# Autodesk Inventor assembly: FullCanAssembly
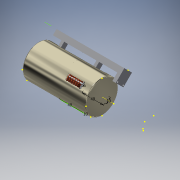
[picture p0: Inventor's stored thumbnail of the model, 180x180]
Saved by Autodesk Inventor 2017.3 (Build 213256000, 256)
## iProperties
Created: 2018-05-23
Part Number: FullCanAssembly
Document SubType Name: Assembly
Designer: Mac
Author: Mac
## Documents named in this file (18)
- C:\Users\Mac\Desktop\UNR Coltrims\eGun Final Design\FullCanAssembly.iam
- C:\Users\Mac\Desktop\UNR Coltrims\eGun Final Design\Ceramic Support.ipt
- C:\Users\Mac\Desktop\UNR Coltrims\eGun Final Design\InnerSleeveBack.ipt
- C:\Users\Mac\Desktop\UNR Coltrims\eGun Final Design\InnerSleeveFront.ipt
- C:\Users\Mac\Desktop\UNR Coltrims\eGun Final Design\13mm Ceramic Spacer.ipt
- C:\Users\Mac\Desktop\UNR Coltrims\eGun Final Design\Pulser Plate.ipt
- C:\Users\Mac\Desktop\UNR Coltrims\eGun Final Design\19mm Ceramic Spacer.ipt
- C:\Users\Mac\Desktop\UNR Coltrims\eGun Final Design\1mm Electrode.ipt
- C:\Users\Mac\Desktop\UNR Coltrims\eGun Final Design\20mm Ceramic Spacer.ipt
- C:\Users\Mac\Desktop\UNR Coltrims\eGun Final Design\3mm Ceramic Spacer.ipt
- C:\Users\Mac\Desktop\UNR Coltrims\eGun Final Design\uMetal Can.ipt
- C:\Users\Mac\Desktop\UNR Coltrims\eGun Final Design\uMetal Can Backside.ipt
- C:\Users\Mac\Desktop\UNR Coltrims\eGun Final Design\4.5mm Ceramic Spacer.ipt
- C:\Users\Mac\Desktop\UNR Coltrims\eGun Final Design\Cathode\Cathode Assembly.iam
- C:\Users\Mac\Desktop\UNR Coltrims\eGun Final Design\Sleeve Endcap.ipt
- C:\Users\Mac\Desktop\UNR Coltrims\eGun Final Design\body rod.ipt
- C:\Users\Mac\Desktop\UNR Coltrims\eGun Final Design\L bracket.ipt
- C:\Users\Mac\Desktop\UNR Coltrims\eGun Final Design\holder square.ipt
## Components (77 placed, 17 different names)
1. Ceramic Support:1 — Mate:1, Mate:2, Mate:3, Mate:4, Mate:5, Mate:6, Mate:7, Mate:8, Mate:9, Mate:16, Mate:17, Mate:19, Mate:20, Mate:22, Mate:23, Mate:24, Mate:25, Mate:26, Mate:27, Mate:34, Mate:35, Mate:37, Mate:38, Mate:39, Mate:40, Mate:41, Mate:42, Mate:49, Mate:50, Mate:52, Mate:53, Mate:54, Mate:55, Mate:56, Mate:57, Mate:64, Mate:65, Mate:67, Mate:68, Mate:69, Mate:70, Mate:71, Mate:72, Mate:79, Mate:80, Mate:82, Mate:83, Mate:84, Mate:85, Mate:86, Mate:87, Mate:94, Mate:95, Mate:97, Mate:98, Mate:99, Mate:100, Mate:101, Mate:102, Mate:109, Mate:110, Mate:112, Mate:113, Mate:114, Mate:115, Mate:116, Mate:117, Mate:124, Mate:125, Mate:127, Mate:128, Mate:129, Mate:130, Mate:131, Mate:132, Mate:139, Mate:140, Mate:142, Mate:143, Mate:144
2. InnerSleeveBack:1 — Mate:145, Mate:146, Mate:147
3. InnerSleeveFront:1 — Mate:1, Mate:2, Mate:3, Mate:10, Mate:11, Mate:12, Mate:13, Mate:14, Mate:15, Mate:148, Mate:149, Mate:150, Mate:151, Flush:1, Flush:2, Flush:3, Flush:4, Mate:152, Mate:153, Mate:161
4. 13mm Ceramic Spacer:1 — Mate:4, Mate:14
5. 13mm Ceramic Spacer:2 — Mate:5, Mate:10
6. 13mm Ceramic Spacer:3 — Mate:6, Mate:11, Mate:18
7. 13mm Ceramic Spacer:4 — Mate:7, Mate:12
8. 13mm Ceramic Spacer:5 — Mate:8, Mate:13
9. 13mm Ceramic Spacer:6 — Mate:9, Mate:15, Mate:21
10. Pulser Plate:1 — Mate:16, Mate:17, Mate:18, Mate:31, Mate:32, Mate:33
11. Pulser Plate:2 — Mate:19, Mate:20, Mate:21, Mate:28, Mate:29, Mate:30
12. 19mm Ceramic Spacer:1 — Mate:22, Mate:29
13. 19mm Ceramic Spacer:2 — Mate:23, Mate:28
14. 19mm Ceramic Spacer:3 — Mate:24, Mate:33, Mate:36
15. 19mm Ceramic Spacer:4 — Mate:25, Mate:32
16. 19mm Ceramic Spacer:5 — Mate:26, Mate:31
17. 19mm Ceramic Spacer:6 — Mate:27, Mate:30
18. 1mm Electrode:1 — Mate:64, Mate:65, Mate:66, Mate:73, Mate:74, Mate:75, Mate:76, Mate:77, Mate:78
19. 1mm Electrode:2 — Mate:34, Mate:35, Mate:36, Mate:43, Mate:44, Mate:45, Mate:46, Mate:47, Mate:48
20. 1mm Electrode:3 — Mate:79, Mate:80, Mate:81, Mate:88, Mate:89, Mate:90, Mate:91, Mate:92, Mate:93
21. 1mm Electrode:4 — Mate:49, Mate:50, Mate:51, Mate:58, Mate:59, Mate:60, Mate:61, Mate:62, Mate:63
22. 1mm Electrode:5 — Mate:109, Mate:110, Mate:111, Mate:118, Mate:119, Mate:120, Mate:121, Mate:122, Mate:123
23. 1mm Electrode:6 — Mate:94, Mate:95, Mate:96, Mate:103, Mate:104, Mate:105, Mate:106, Mate:107, Mate:108
24. 20mm Ceramic Spacer:1 — Mate:42, Mate:48
25. 20mm Ceramic Spacer:2 — Mate:41, Mate:47
26. 20mm Ceramic Spacer:3 — Mate:40, Mate:46
27. 20mm Ceramic Spacer:4 — Mate:39, Mate:45
28. 20mm Ceramic Spacer:5 — Mate:38, Mate:44
29. 20mm Ceramic Spacer:6 — Mate:37, Mate:43, Mate:51
30. 3mm Ceramic Spacer:1 — Mate:52, Mate:61
31. 3mm Ceramic Spacer:2 — Mate:53, Mate:62
32. 3mm Ceramic Spacer:3 — Mate:54, Mate:63
33. 3mm Ceramic Spacer:4 — Mate:55, Mate:58
34. 3mm Ceramic Spacer:5 — Mate:56, Mate:59
35. 3mm Ceramic Spacer:6 — Mate:57, Mate:60, Mate:66
36. 3mm Ceramic Spacer:7 — Mate:87, Mate:91
37. 3mm Ceramic Spacer:8 — Mate:86, Mate:90
38. 3mm Ceramic Spacer:9 — Mate:85, Mate:89
39. 3mm Ceramic Spacer:10 — Mate:84, Mate:88
40. 3mm Ceramic Spacer:11 — Mate:83, Mate:93
41. 3mm Ceramic Spacer:12 — Mate:82, Mate:92, Mate:96
42. 3mm Ceramic Spacer:13 — Mate:102, Mate:107
43. 3mm Ceramic Spacer:14 — Mate:101, Mate:106
44. 3mm Ceramic Spacer:15 — Mate:100, Mate:105
45. 3mm Ceramic Spacer:16 — Mate:99, Mate:104
46. 3mm Ceramic Spacer:17 — Mate:98, Mate:103, Mate:111
47. 3mm Ceramic Spacer:18 — Mate:97, Mate:108
48. 3mm Ceramic Spacer:19 — Mate:112, Mate:120
49. 3mm Ceramic Spacer:20 — Mate:113, Mate:118
50. 3mm Ceramic Spacer:21 — Mate:114, Mate:119
51. 3mm Ceramic Spacer:22 — Mate:115, Mate:123
52. 3mm Ceramic Spacer:23 — Mate:116, Mate:122, Mate:126
53. 3mm Ceramic Spacer:24 — Mate:117, Mate:121
54. 3mm Ceramic Spacer:25 — Mate:67, Mate:73
55. 3mm Ceramic Spacer:26 — Mate:72, Mate:74, Mate:81
56. 3mm Ceramic Spacer:27 — Mate:71, Mate:78
57. 3mm Ceramic Spacer:28 — Mate:70, Mate:77
58. 3mm Ceramic Spacer:29 — Mate:69, Mate:76
59. 3mm Ceramic Spacer:30 — Mate:68, Mate:75
60. uMetal Can:1 — Mate:152, Mate:153, Mate:154, Flush:5, Angle:1, Mate:161, Mate:162, Mate:163
61. uMetal Can Backside:1 — Mate:154, Flush:5, Mate:162
62. 1mm Electrode:7 — Mate:124, Mate:125, Mate:126, Mate:133, Mate:134, Mate:135, Mate:136, Mate:137, Mate:138
63. 4.5mm Ceramic Spacer:1 — Mate:127, Mate:137
64. 4.5mm Ceramic Spacer:2 — Mate:128, Mate:133
65. 4.5mm Ceramic Spacer:3 — Mate:129, Mate:134
66. 4.5mm Ceramic Spacer:4 — Mate:130, Mate:135
67. 4.5mm Ceramic Spacer:5 — Mate:131, Mate:136
68. 4.5mm Ceramic Spacer:6 — Mate:132, Mate:138, Mate:141
69. Cathode Assembly:1 [sub-assembly] — Mate:139, Mate:140, Mate:141
70. Sleeve Endcap:1 — Mate:142, Mate:143, Mate:144, Mate:145, Mate:146, Mate:147
71. body rod:1 — Mate:148, Flush:3
72. body rod:2 — Mate:149, Flush:1, Mate:155, Mate:157
73. body rod:3 — Mate:150, Flush:4
74. body rod:4 — Mate:151, Flush:2
75. L bracket:1 — Mate:158, Mate:159, Mate:160
76. holder square:1 — Mate:155, Flush:6, Mate:158, Mate:159, Angle:1, Mate:163
77. holder square:2 — Mate:157, Flush:6, Mate:160
## Relationships (169: Mate 162, Flush 6, Angle 1)
- Mate:1: Ceramic Support:1 ↔ InnerSleeveFront:1
- Mate:2: Ceramic Support:1 ↔ InnerSleeveFront:1
- Mate:3: Ceramic Support:1 ↔ InnerSleeveFront:1
- Mate:4: Ceramic Support:1 ↔ 13mm Ceramic Spacer:1
- Mate:5: Ceramic Support:1 ↔ 13mm Ceramic Spacer:2
- Mate:6: Ceramic Support:1 ↔ 13mm Ceramic Spacer:3
- Mate:7: Ceramic Support:1 ↔ 13mm Ceramic Spacer:4
- Mate:8: Ceramic Support:1 ↔ 13mm Ceramic Spacer:5
- Mate:9: Ceramic Support:1 ↔ 13mm Ceramic Spacer:6
- Mate:10: InnerSleeveFront:1 ↔ 13mm Ceramic Spacer:2
- Mate:11: InnerSleeveFront:1 ↔ 13mm Ceramic Spacer:3
- Mate:12: InnerSleeveFront:1 ↔ 13mm Ceramic Spacer:4
- Mate:13: InnerSleeveFront:1 ↔ 13mm Ceramic Spacer:5
- Mate:14: InnerSleeveFront:1 ↔ 13mm Ceramic Spacer:1
- Mate:15: InnerSleeveFront:1 ↔ 13mm Ceramic Spacer:6
- Mate:16: Ceramic Support:1 ↔ Pulser Plate:1
- Mate:17: Ceramic Support:1 ↔ Pulser Plate:1
- Mate:18: 13mm Ceramic Spacer:3 ↔ Pulser Plate:1
- Mate:19: Ceramic Support:1 ↔ Pulser Plate:2
- Mate:20: Ceramic Support:1 ↔ Pulser Plate:2
- Mate:21: 13mm Ceramic Spacer:6 ↔ Pulser Plate:2
- Mate:22: Ceramic Support:1 ↔ 19mm Ceramic Spacer:1
- Mate:23: Ceramic Support:1 ↔ 19mm Ceramic Spacer:2
- Mate:24: Ceramic Support:1 ↔ 19mm Ceramic Spacer:3
- Mate:25: Ceramic Support:1 ↔ 19mm Ceramic Spacer:4
- Mate:26: Ceramic Support:1 ↔ 19mm Ceramic Spacer:5
- Mate:27: Ceramic Support:1 ↔ 19mm Ceramic Spacer:6
- Mate:28: Pulser Plate:2 ↔ 19mm Ceramic Spacer:2
- Mate:29: Pulser Plate:2 ↔ 19mm Ceramic Spacer:1
- Mate:30: Pulser Plate:2 ↔ 19mm Ceramic Spacer:6
- Mate:31: Pulser Plate:1 ↔ 19mm Ceramic Spacer:5
- Mate:32: Pulser Plate:1 ↔ 19mm Ceramic Spacer:4
- Mate:33: Pulser Plate:1 ↔ 19mm Ceramic Spacer:3
- Mate:34: Ceramic Support:1 ↔ 1mm Electrode:2
- Mate:35: Ceramic Support:1 ↔ 1mm Electrode:2
- Mate:36: 19mm Ceramic Spacer:3 ↔ 1mm Electrode:2
- Mate:37: Ceramic Support:1 ↔ 20mm Ceramic Spacer:6
- Mate:38: Ceramic Support:1 ↔ 20mm Ceramic Spacer:5
- Mate:39: Ceramic Support:1 ↔ 20mm Ceramic Spacer:4
- Mate:40: Ceramic Support:1 ↔ 20mm Ceramic Spacer:3
- Mate:41: Ceramic Support:1 ↔ 20mm Ceramic Spacer:2
- Mate:42: Ceramic Support:1 ↔ 20mm Ceramic Spacer:1
- Mate:43: 1mm Electrode:2 ↔ 20mm Ceramic Spacer:6
- Mate:44: 1mm Electrode:2 ↔ 20mm Ceramic Spacer:5
- Mate:45: 1mm Electrode:2 ↔ 20mm Ceramic Spacer:4
- Mate:46: 1mm Electrode:2 ↔ 20mm Ceramic Spacer:3
- Mate:47: 1mm Electrode:2 ↔ 20mm Ceramic Spacer:2
- Mate:48: 1mm Electrode:2 ↔ 20mm Ceramic Spacer:1
- Mate:49: Ceramic Support:1 ↔ 1mm Electrode:4
- Mate:50: Ceramic Support:1 ↔ 1mm Electrode:4
- Mate:51: 1mm Electrode:4 ↔ 20mm Ceramic Spacer:6
- Mate:52: Ceramic Support:1 ↔ 3mm Ceramic Spacer:1
- Mate:53: Ceramic Support:1 ↔ 3mm Ceramic Spacer:2
- Mate:54: Ceramic Support:1 ↔ 3mm Ceramic Spacer:3
- Mate:55: Ceramic Support:1 ↔ 3mm Ceramic Spacer:4
- Mate:56: Ceramic Support:1 ↔ 3mm Ceramic Spacer:5
- Mate:57: Ceramic Support:1 ↔ 3mm Ceramic Spacer:6
- Mate:58: 1mm Electrode:4 ↔ 3mm Ceramic Spacer:4
- Mate:59: 1mm Electrode:4 ↔ 3mm Ceramic Spacer:5
- Mate:60: 1mm Electrode:4 ↔ 3mm Ceramic Spacer:6
- Mate:61: 1mm Electrode:4 ↔ 3mm Ceramic Spacer:1
- Mate:62: 1mm Electrode:4 ↔ 3mm Ceramic Spacer:2
- Mate:63: 1mm Electrode:4 ↔ 3mm Ceramic Spacer:3
- Mate:64: Ceramic Support:1 ↔ 1mm Electrode:1
- Mate:65: Ceramic Support:1 ↔ 1mm Electrode:1
- Mate:66: 1mm Electrode:1 ↔ 3mm Ceramic Spacer:6
- Mate:67: Ceramic Support:1 ↔ 3mm Ceramic Spacer:25
- Mate:68: Ceramic Support:1 ↔ 3mm Ceramic Spacer:30
- Mate:69: Ceramic Support:1 ↔ 3mm Ceramic Spacer:29
- Mate:70: Ceramic Support:1 ↔ 3mm Ceramic Spacer:28
- Mate:71: Ceramic Support:1 ↔ 3mm Ceramic Spacer:27
- Mate:72: Ceramic Support:1 ↔ 3mm Ceramic Spacer:26
- Mate:73: 1mm Electrode:1 ↔ 3mm Ceramic Spacer:25
- Mate:74: 1mm Electrode:1 ↔ 3mm Ceramic Spacer:26
- Mate:75: 1mm Electrode:1 ↔ 3mm Ceramic Spacer:30
- Mate:76: 1mm Electrode:1 ↔ 3mm Ceramic Spacer:29
- Mate:77: 1mm Electrode:1 ↔ 3mm Ceramic Spacer:28
- Mate:78: 1mm Electrode:1 ↔ 3mm Ceramic Spacer:27
- Mate:79: Ceramic Support:1 ↔ 1mm Electrode:3
- Mate:80: Ceramic Support:1 ↔ 1mm Electrode:3
- Mate:81: 1mm Electrode:3 ↔ 3mm Ceramic Spacer:26
- Mate:82: Ceramic Support:1 ↔ 3mm Ceramic Spacer:12
- Mate:83: Ceramic Support:1 ↔ 3mm Ceramic Spacer:11
- Mate:84: Ceramic Support:1 ↔ 3mm Ceramic Spacer:10
- Mate:85: Ceramic Support:1 ↔ 3mm Ceramic Spacer:9
- Mate:86: Ceramic Support:1 ↔ 3mm Ceramic Spacer:8
- Mate:87: Ceramic Support:1 ↔ 3mm Ceramic Spacer:7
- Mate:88: 1mm Electrode:3 ↔ 3mm Ceramic Spacer:10
- Mate:89: 1mm Electrode:3 ↔ 3mm Ceramic Spacer:9
- Mate:90: 1mm Electrode:3 ↔ 3mm Ceramic Spacer:8
- Mate:91: 1mm Electrode:3 ↔ 3mm Ceramic Spacer:7
- Mate:92: 1mm Electrode:3 ↔ 3mm Ceramic Spacer:12
- Mate:93: 1mm Electrode:3 ↔ 3mm Ceramic Spacer:11
- Mate:94: Ceramic Support:1 ↔ 1mm Electrode:6
- Mate:95: Ceramic Support:1 ↔ 1mm Electrode:6
- Mate:96: 1mm Electrode:6 ↔ 3mm Ceramic Spacer:12
- Mate:97: Ceramic Support:1 ↔ 3mm Ceramic Spacer:18
- Mate:98: Ceramic Support:1 ↔ 3mm Ceramic Spacer:17
- Mate:99: Ceramic Support:1 ↔ 3mm Ceramic Spacer:16
- Mate:100: Ceramic Support:1 ↔ 3mm Ceramic Spacer:15
- Mate:101: Ceramic Support:1 ↔ 3mm Ceramic Spacer:14
- Mate:102: Ceramic Support:1 ↔ 3mm Ceramic Spacer:13
- Mate:103: 1mm Electrode:6 ↔ 3mm Ceramic Spacer:17
- Mate:104: 1mm Electrode:6 ↔ 3mm Ceramic Spacer:16
- Mate:105: 1mm Electrode:6 ↔ 3mm Ceramic Spacer:15
- Mate:106: 1mm Electrode:6 ↔ 3mm Ceramic Spacer:14
- Mate:107: 1mm Electrode:6 ↔ 3mm Ceramic Spacer:13
- Mate:108: 1mm Electrode:6 ↔ 3mm Ceramic Spacer:18
- Mate:109: Ceramic Support:1 ↔ 1mm Electrode:5
- Mate:110: Ceramic Support:1 ↔ 1mm Electrode:5
- Mate:111: 1mm Electrode:5 ↔ 3mm Ceramic Spacer:17
- Mate:112: Ceramic Support:1 ↔ 3mm Ceramic Spacer:19
- Mate:113: Ceramic Support:1 ↔ 3mm Ceramic Spacer:20
- Mate:114: Ceramic Support:1 ↔ 3mm Ceramic Spacer:21
- Mate:115: Ceramic Support:1 ↔ 3mm Ceramic Spacer:22
- Mate:116: Ceramic Support:1 ↔ 3mm Ceramic Spacer:23
- Mate:117: Ceramic Support:1 ↔ 3mm Ceramic Spacer:24
- Mate:118: 1mm Electrode:5 ↔ 3mm Ceramic Spacer:20
- Mate:119: 1mm Electrode:5 ↔ 3mm Ceramic Spacer:21
- Mate:120: 1mm Electrode:5 ↔ 3mm Ceramic Spacer:19
- Mate:121: 1mm Electrode:5 ↔ 3mm Ceramic Spacer:24
- Mate:122: 1mm Electrode:5 ↔ 3mm Ceramic Spacer:23
- Mate:123: 1mm Electrode:5 ↔ 3mm Ceramic Spacer:22
- Mate:124: Ceramic Support:1 ↔ 1mm Electrode:7
- Mate:125: Ceramic Support:1 ↔ 1mm Electrode:7
- Mate:126: 3mm Ceramic Spacer:23 ↔ 1mm Electrode:7
- Mate:127: Ceramic Support:1 ↔ 4.5mm Ceramic Spacer:1
- Mate:128: Ceramic Support:1 ↔ 4.5mm Ceramic Spacer:2
- Mate:129: Ceramic Support:1 ↔ 4.5mm Ceramic Spacer:3
- Mate:130: Ceramic Support:1 ↔ 4.5mm Ceramic Spacer:4
- Mate:131: Ceramic Support:1 ↔ 4.5mm Ceramic Spacer:5
- Mate:132: Ceramic Support:1 ↔ 4.5mm Ceramic Spacer:6
- Mate:133: 1mm Electrode:7 ↔ 4.5mm Ceramic Spacer:2
- Mate:134: 1mm Electrode:7 ↔ 4.5mm Ceramic Spacer:3
- Mate:135: 1mm Electrode:7 ↔ 4.5mm Ceramic Spacer:4
- Mate:136: 1mm Electrode:7 ↔ 4.5mm Ceramic Spacer:5
- Mate:137: 1mm Electrode:7 ↔ 4.5mm Ceramic Spacer:1
- Mate:138: 1mm Electrode:7 ↔ 4.5mm Ceramic Spacer:6
- Mate:139: Ceramic Support:1 ↔ Cathode Assembly:1
- Mate:140: Ceramic Support:1 ↔ Cathode Assembly:1
- Mate:141: 4.5mm Ceramic Spacer:6 ↔ Cathode Assembly:1
- Mate:142: Ceramic Support:1 ↔ Sleeve Endcap:1
- Mate:143: Ceramic Support:1 ↔ Sleeve Endcap:1
- Mate:144: Ceramic Support:1 ↔ Sleeve Endcap:1
- Mate:145: InnerSleeveBack:1 ↔ Sleeve Endcap:1
- Mate:146: InnerSleeveBack:1 ↔ Sleeve Endcap:1
- Mate:147: InnerSleeveBack:1 ↔ Sleeve Endcap:1
- Mate:148: InnerSleeveFront:1 ↔ body rod:1
- Mate:149: InnerSleeveFront:1 ↔ body rod:2
- Mate:150: InnerSleeveFront:1 ↔ body rod:3
- Mate:151: InnerSleeveFront:1 ↔ body rod:4
- Flush:1: InnerSleeveFront:1 ↔ body rod:2
- Flush:2: InnerSleeveFront:1 ↔ body rod:4
- Flush:3: InnerSleeveFront:1 ↔ body rod:1
- Flush:4: InnerSleeveFront:1 ↔ body rod:3
- Mate:152: InnerSleeveFront:1 ↔ uMetal Can:1
- Mate:153: InnerSleeveFront:1 ↔ uMetal Can:1
- Mate:154: uMetal Can:1 ↔ uMetal Can Backside:1
- Flush:5: uMetal Can:1 ↔ uMetal Can Backside:1
- Mate:155: body rod:2 ↔ holder square:1
- Mate:157: body rod:2 ↔ holder square:2
- Flush:6: holder square:1 ↔ holder square:2
- Mate:158: L bracket:1 ↔ holder square:1
- Mate:159: L bracket:1 ↔ holder square:1
- Mate:160: L bracket:1 ↔ holder square:2
- Angle:1 (180 deg): uMetal Can:1 ↔ holder square:1
- Mate:161: InnerSleeveFront:1 ↔ uMetal Can:1
- Mate:162: uMetal Can:1 ↔ uMetal Can Backside:1
- Mate:163 (1.5875 mm): uMetal Can:1 ↔ holder square:1
